# Autodesk Inventor assembly: motorAssembly
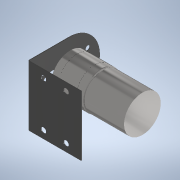
[picture p0: Inventor's stored thumbnail of the model, 180x180]
Saved by Autodesk Inventor 2020 (Build 240168000, 168)
## iProperties
Created: 2022-07-22
Part Number: motorAssembly
Document SubType Name: Assembly
Designer: iPICLab4
Author: iPICLab4
## Documents named in this file (3)
- C:\Users\karimi2\Documents\PROJECT\src\motorAssembly.iam
- C:\Users\karimi2\Documents\PROJECT\src\GearedDCmotor.ipt
- C:\Users\karimi2\Documents\PROJECT\src\motorBracket.ipt
## Components (2 placed, 2 different names)
1. GearedDCmotor:1 — Mate:1
2. motorBracket:1 — Mate:1
## Relationships (1: Mate 1)
- Mate:1: GearedDCmotor:1 ↔ motorBracket:1
